# Autodesk Inventor assembly: Z_Bed
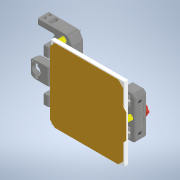
[picture p0: Inventor's stored thumbnail of the model, 180x180]
Saved by Autodesk Inventor 2022 (Build 260153000, 153)
## iProperties
Created: 2021-11-24
Part Number: Z_Bed
Document SubType Name: Assembly
Designer: yuto6
Author: yuto6
## Documents named in this file (12)
- C:\Users\yuto6\Documents\My3DPrinter\CAD\Asm\Z_Bed.iam
- C:\Users\yuto6\Documents\My3DPrinter\CAD\Parts\Build Plate.iam
- C:\Users\yuto6\Documents\My3DPrinter\CAD\Parts\yellow dia spring.step.ipt
- C:\Users\yuto6\Documents\My3DPrinter\CAD\Parts\Front_Bed_Mount.step.ipt
- C:\Users\yuto6\Documents\My3DPrinter\CAD\Parts\Thumb_Nut.step.ipt
- C:\Users\yuto6\Documents\My3DPrinter\CAD\Parts\M3 Threaded Insert.step.ipt
- C:\Users\yuto6\Documents\My3DPrinter\CAD\Parts\HFS3-1515-100.ipt
- C:\Users\yuto6\Documents\My3DPrinter\CAD\Parts\M3x12 BHCS.step.ipt
- C:\Users\yuto6\Documents\My3DPrinter\CAD\Parts\M3x8 BHCS-1.step.ipt
- C:\Users\yuto6\Documents\My3DPrinter\CAD\Parts\t8 nut block-1.step.ipt
- C:\Users\yuto6\Documents\My3DPrinter\CAD\Parts\Rear_Bed_Mount_Left.step.ipt
- C:\Users\yuto6\Documents\My3DPrinter\CAD\Parts\Rear_Bed_Mount_Right.step.ipt
## Components (17 placed, 11 different names)
1. Build Plate:1 [sub-assembly] — メイト:1, メイト:2, メイト:3, メイト:4, フラッシュ:1, メイト:6, 角度:1, メイト:24, メイト:26
2. yellow dia spring.step:1 — メイト:1
3. yellow dia spring.step:2 — メイト:3
4. yellow dia spring.step:3 — メイト:2
5. Front_Bed_Mount.step:1 — メイト:4, フラッシュ:1, メイト:7, メイト:8, 角度:1, メイト:9, メイト:10, メイト:11, メイト:12, メイト:13, メイト:15, メイト:16, メイト:17, メイト:18, メイト:19, メイト:20, メイト:21, メイト:22
6. Thumb_Nut.step:1 — メイト:5, フラッシュ:2, メイト:7
7. M3 Threaded Insert.step:1 — メイト:5, フラッシュ:2, メイト:6
8. HFS3-1515-100:1 — メイト:10, メイト:11, メイト:12, フラッシュ:3
9. HFS3-1515-100:2 — メイト:8, メイト:9, メイト:13, メイト:14
10. HFS3-1515-100:3 — メイト:14, フラッシュ:3, フラッシュ:4, メイト:23, フラッシュ:5, 角度:2, メイト:25, 角度:3, メイト:27
11. M3x12 BHCS.step:1 — メイト:15, メイト:18
12. M3x12 BHCS.step:2 — メイト:16, メイト:17
13. M3x8 BHCS-1.step:1 — メイト:20, メイト:22
14. M3x8 BHCS-1.step:2 — メイト:19, メイト:21
15. t8 nut block-1.step:1 — フラッシュ:4, メイト:23, フラッシュ:5
16. Rear_Bed_Mount_Left.step:1 — メイト:24, 角度:2, メイト:25
17. Rear_Bed_Mount_Right.step:1 — メイト:26, 角度:3, メイト:27
## Relationships (35: Mate 27, Flush 5, Angle 3)
- メイト:1 [Mate]: Build Plate:1 ↔ yellow dia spring.step:1
- メイト:2 [Mate]: Build Plate:1 ↔ yellow dia spring.step:3
- メイト:3 [Mate]: Build Plate:1 ↔ yellow dia spring.step:2
- メイト:4 [Mate]: Build Plate:1 ↔ Front_Bed_Mount.step:1
- フラッシュ:1 [Flush] (9.35 mm): Build Plate:1 ↔ Front_Bed_Mount.step:1
- メイト:5 [Mate]: Thumb_Nut.step:1 ↔ M3 Threaded Insert.step:1
- フラッシュ:2 [Flush]: Thumb_Nut.step:1 ↔ M3 Threaded Insert.step:1
- メイト:6 [Mate]: Build Plate:1 ↔ M3 Threaded Insert.step:1
- メイト:7 [Mate]: Front_Bed_Mount.step:1 ↔ Thumb_Nut.step:1
- メイト:8 [Mate]: Front_Bed_Mount.step:1 ↔ HFS3-1515-100:2
- 角度:1 [Angle] (0 deg): Build Plate:1 ↔ Front_Bed_Mount.step:1
- メイト:9 [Mate]: Front_Bed_Mount.step:1 ↔ HFS3-1515-100:2
- メイト:10 [Mate]: Front_Bed_Mount.step:1 ↔ HFS3-1515-100:1
- メイト:11 [Mate]: Front_Bed_Mount.step:1 ↔ HFS3-1515-100:1
- メイト:12 [Mate]: Front_Bed_Mount.step:1 ↔ HFS3-1515-100:1
- メイト:13 [Mate]: Front_Bed_Mount.step:1 ↔ HFS3-1515-100:2
- メイト:14 [Mate]: HFS3-1515-100:2 ↔ HFS3-1515-100:3
- メイト:15 [Mate]: Front_Bed_Mount.step:1 ↔ M3x12 BHCS.step:1
- メイト:16 [Mate]: Front_Bed_Mount.step:1 ↔ M3x12 BHCS.step:2
- メイト:17 [Mate]: Front_Bed_Mount.step:1 ↔ M3x12 BHCS.step:2
- メイト:18 [Mate]: Front_Bed_Mount.step:1 ↔ M3x12 BHCS.step:1
- メイト:19 [Mate]: Front_Bed_Mount.step:1 ↔ M3x8 BHCS-1.step:2
- メイト:20 [Mate]: Front_Bed_Mount.step:1 ↔ M3x8 BHCS-1.step:1
- メイト:21 [Mate]: Front_Bed_Mount.step:1 ↔ M3x8 BHCS-1.step:2
- メイト:22 [Mate]: Front_Bed_Mount.step:1 ↔ M3x8 BHCS-1.step:1
- フラッシュ:3 [Flush]: HFS3-1515-100:1 ↔ HFS3-1515-100:3
- フラッシュ:4 [Flush]: HFS3-1515-100:3 ↔ t8 nut block-1.step:1
- メイト:23 [Mate]: HFS3-1515-100:3 ↔ t8 nut block-1.step:1
- フラッシュ:5 [Flush] (36 mm): HFS3-1515-100:3 ↔ t8 nut block-1.step:1
- メイト:24 [Mate]: Build Plate:1 ↔ Rear_Bed_Mount_Left.step:1
- 角度:2 [Angle] (0 deg): HFS3-1515-100:3 ↔ Rear_Bed_Mount_Left.step:1
- メイト:25 [Mate]: HFS3-1515-100:3 ↔ Rear_Bed_Mount_Left.step:1
- メイト:26 [Mate]: Build Plate:1 ↔ Rear_Bed_Mount_Right.step:1
- 角度:3 [Angle] (0 deg): HFS3-1515-100:3 ↔ Rear_Bed_Mount_Right.step:1
- メイト:27 [Mate]: HFS3-1515-100:3 ↔ Rear_Bed_Mount_Right.step:1
